# Autodesk Inventor assembly: HS 36T Gear, No Insert1
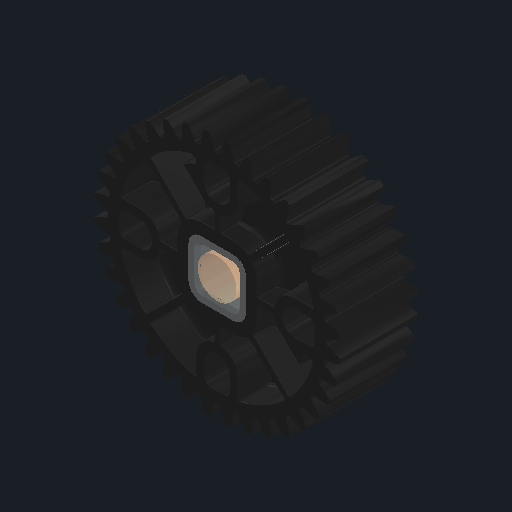
[picture p0: Inventor's stored thumbnail of the model, 512x512]
Saved by Autodesk Inventor 2025 (Build 290162000, 162)
## iProperties
Created: 2022-08-02
Part Number: HS 36T Gear, No Insert1
Document SubType Name: Assembly
Designer: Averey Ku
Author: ylu12
## Documents named in this file (2)
- D:\VEX\High Stakes\CAD\V4\Chassis\Drivebay Right\HS 36T Gear, No Insert1.iam
- D:\VEX\High Stakes\CAD\V4\Chassis\Drivebay Right\HS 36T Gear, No Insert1.ipt
## Components (1 placed, 1 different names)
1. HS 36T Gear, No Insert1:1 — Flush:5, Mate:9, Mate:10
## Relationships (3: Mate 2, Flush 1)
- Flush:5: HS 36T Gear, No Insert1:1
- Mate:9: HS 36T Gear, No Insert1:1
- Mate:10: HS 36T Gear, No Insert1:1
